# Autodesk Inventor assembly: cannon
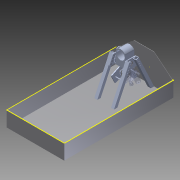
[picture p0: Inventor's stored thumbnail of the model, 180x180]
Saved by Autodesk Inventor 2012 (Build 160160000, 160)
## iProperties
Created: 2012-04-26
Part Number: cannon
Document SubType Name: Assembly
Designer: Robotics
Author: Robotics
## Documents named in this file (4)
- Z:\Old CAD Files\CAD SolidWorks\T-Shirt Cannon\cannon.iam
- C:\Users\robotics\Dropbox\CAD Inventor\Preseason 2012-13\cannon chasis.ipt
- C:\Users\robotics\Dropbox\CAD Inventor\Preseason 2012-13\Imported Components\T-Shirt Cannon\T-Shirt Cannon.iam
- Z:\Old CAD Files\CAD SolidWorks\T-Shirt Cannon\Cover_Back.ipt
## Components (3 placed, 3 different names)
1. cannon chasis:1 — Mate:1, Mate:2, Mate:3, Mate:4
2. T-Shirt Cannon:1 [sub-assembly] — Mate:1, Mate:2
3. Cover_Back:1 — Mate:3, Mate:4
## Relationships (4: Mate 4)
- Mate:1: cannon chasis:1 ↔ T-Shirt Cannon:1
- Mate:2: cannon chasis:1 ↔ T-Shirt Cannon:1
- Mate:3: cannon chasis:1 ↔ Cover_Back:1
- Mate:4: cannon chasis:1 ↔ Cover_Back:1
